# Autodesk Inventor assembly: sip_n_puff_assembly
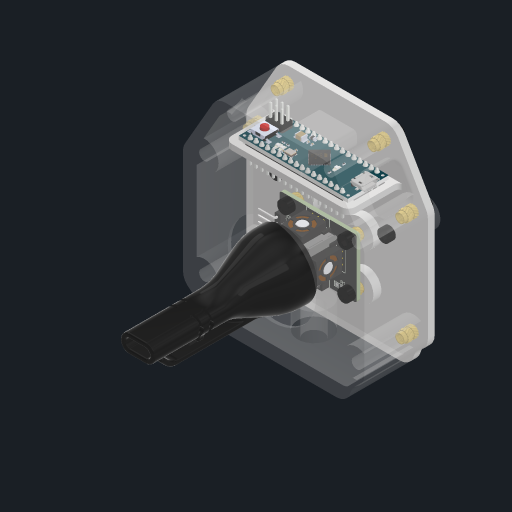
[picture p0: Inventor's stored thumbnail of the model, 512x512]
Saved by Autodesk Inventor 2024 (Build 280153000, 153)
## iProperties
Created: 2025-03-05
Part Number: sip_n_puff_assembly
Document SubType Name: Assembly
Designer: colel
Author: colel
## Documents named in this file (10)
- C:\Users\colel\OneDrive\Desktop\Desktop Folders\Dorm Projects\sip_n_puff_project\sip_n_puff_assembly.iam
- C:\Users\colel\OneDrive\Desktop\Desktop Folders\Dorm Projects\sip_n_puff_project\full_joystick.iam
- C:\Users\colel\OneDrive\Desktop\Desktop Folders\Dorm Projects\sip_n_puff_project\3mm x 6mmL screw.ipt
- C:\Users\colel\OneDrive\Desktop\Desktop Folders\Dorm Projects\sip_n_puff_project\Insert M3 D5 L5mm.ipt
- C:\Users\colel\OneDrive\Desktop\Desktop Folders\Dorm Projects\sip_n_puff_project\mouthpiece.ipt
- C:\Users\colel\OneDrive\Desktop\Desktop Folders\Dorm Projects\sip_n_puff_project\6X6X4.3_BUTTON.ipt
- C:\Users\colel\OneDrive\Desktop\Desktop Folders\Dorm Projects\sip_n_puff_project\Sip_n_box.ipt
- C:\Users\colel\OneDrive\Desktop\Desktop Folders\Dorm Projects\sip_n_puff_project\sip_n_cap.ipt
- C:\Users\colel\OneDrive\Desktop\Desktop Folders\Dorm Projects\sip_n_puff_project\pressure_housing.ipt
- C:\Users\colel\OneDrive\Desktop\Desktop Folders\Dorm Projects\Arduino Stuff\ARDUINO MICRO.iam
## Components (31 placed, 9 different names)
1. full_joystick:1 [sub-assembly] — Mate:1, Mate:2, Mate:3, Mate:4, Mate:5, Mate:6, Mate:7, Mate:8, Mate:10, Mate:14, Mate:15, Mate:16, Mate:21, Mate:22, Tangent:1
2. 3mm x 6mmL screw:1 — Mate:1, Mate:2, Mate:12
3. 3mm x 6mmL screw:2 — Mate:7, Mate:8, Mate:9
4. 3mm x 6mmL screw:3 — Mate:5, Mate:6, Mate:13
5. 3mm x 6mmL screw:4 — Mate:3, Mate:4, Mate:11
6. Insert M3 D5 L5mm:1 — Mate:9, Mate:10
7. Insert M3 D5 L5mm:2 — Mate:12, Mate:16, Mate:25
8. Insert M3 D5 L5mm:3 — Mate:13, Mate:15, Mate:24, Mate:26
9. Insert M3 D5 L5mm:4 — Mate:11, Mate:14
10. mouthpiece:1 — Mate:19, Mate:20, Mate:21, Mate:22, Tangent:1, Mate:23
11. 6X6X4.3_BUTTON:1 — Mate:19, Mate:20, Mate:23
12. Sip_n_box:1 — Mate:24, Mate:25, Mate:26, Mate:36, Mate:37, Mate:44, Mate:45, Mate:46, Mate:47, Mate:49, Mate:50, Mate:51, Mate:52, Mate:53, Mate:54, Mate:55, Mate:56, Mate:57, Mate:58, Mate:59, Mate:60, Mate:65, Mate:66, Mate:67, Mate:68, Mate:69
13. sip_n_cap:1 — Mate:30, Flush:1, Mate:31, Flush:2, Mate:32, Flush:3, Mate:33, Flush:4, Mate:34, Flush:5, Mate:35, Flush:6, Mate:69
14. Insert M3 D5 L5mm:7 — Mate:33, Flush:4, Mate:36
15. Insert M3 D5 L5mm:8 — Mate:34, Flush:5
16. Insert M3 D5 L5mm:9 — Mate:35, Flush:6
17. Insert M3 D5 L5mm:10 — Mate:32, Flush:3
18. Insert M3 D5 L5mm:11 — Mate:31, Flush:2
19. Insert M3 D5 L5mm:12 — Mate:30, Flush:1, Mate:37
20. Insert M3 D5 L5mm:13 — Mate:62, Flush:8
21. Insert M3 D5 L5mm:16 — Mate:61, Flush:7
22. 3mm x 6mmL screw:5 — Mate:46, Mate:47, Mate:63
23. 3mm x 6mmL screw:6 — Mate:44, Mate:45, Mate:64
24. 3mm x 6mmL screw:7 — Mate:49, Mate:50
25. 3mm x 6mmL screw:8 — Mate:55, Mate:56
26. 3mm x 6mmL screw:9 — Mate:57, Mate:58
27. 3mm x 6mmL screw:10 — Mate:59, Mate:60
28. 3mm x 6mmL screw:11 — Mate:53, Mate:54
29. 3mm x 6mmL screw:12 — Mate:51, Mate:52
30. pressure_housing:1 — Mate:61, Flush:7, Mate:62, Flush:8, Mate:63, Mate:64, Mate:65
31. ARDUINO MICRO:1 [sub-assembly] — Mate:66, Mate:67, Mate:68
## Relationships (66: Mate 57, Flush 8, Tangent 1)
- Mate:1: full_joystick:1 ↔ 3mm x 6mmL screw:1
- Mate:2: full_joystick:1 ↔ 3mm x 6mmL screw:1
- Mate:3: full_joystick:1 ↔ 3mm x 6mmL screw:4
- Mate:4: full_joystick:1 ↔ 3mm x 6mmL screw:4
- Mate:5: full_joystick:1 ↔ 3mm x 6mmL screw:3
- Mate:6: full_joystick:1 ↔ 3mm x 6mmL screw:3
- Mate:7: full_joystick:1 ↔ 3mm x 6mmL screw:2
- Mate:8: full_joystick:1 ↔ 3mm x 6mmL screw:2
- Mate:9: 3mm x 6mmL screw:2 ↔ Insert M3 D5 L5mm:1
- Mate:10: full_joystick:1 ↔ Insert M3 D5 L5mm:1
- Mate:11: 3mm x 6mmL screw:4 ↔ Insert M3 D5 L5mm:4
- Mate:12: 3mm x 6mmL screw:1 ↔ Insert M3 D5 L5mm:2
- Mate:13: 3mm x 6mmL screw:3 ↔ Insert M3 D5 L5mm:3
- Mate:14: full_joystick:1 ↔ Insert M3 D5 L5mm:4
- Mate:15: full_joystick:1 ↔ Insert M3 D5 L5mm:3
- Mate:16: full_joystick:1 ↔ Insert M3 D5 L5mm:2
- Mate:19 (0.25 mm): mouthpiece:1 ↔ 6X6X4.3_BUTTON:1
- Mate:20 (0.25 mm): mouthpiece:1 ↔ 6X6X4.3_BUTTON:1
- Mate:21 (0.25 mm): full_joystick:1 ↔ mouthpiece:1
- Mate:22 (0.25 mm): full_joystick:1 ↔ mouthpiece:1
- Tangent:1: full_joystick:1 ↔ mouthpiece:1
- Mate:23: mouthpiece:1 ↔ 6X6X4.3_BUTTON:1
- Mate:24: Insert M3 D5 L5mm:3 ↔ Sip_n_box:1
- Mate:25: Insert M3 D5 L5mm:2 ↔ Sip_n_box:1
- Mate:26: Insert M3 D5 L5mm:3 ↔ Sip_n_box:1
- Mate:30: sip_n_cap:1 ↔ Insert M3 D5 L5mm:12
- Flush:1: sip_n_cap:1 ↔ Insert M3 D5 L5mm:12
- Mate:31: sip_n_cap:1 ↔ Insert M3 D5 L5mm:11
- Flush:2: sip_n_cap:1 ↔ Insert M3 D5 L5mm:11
- Mate:32: sip_n_cap:1 ↔ Insert M3 D5 L5mm:10
- Flush:3: sip_n_cap:1 ↔ Insert M3 D5 L5mm:10
- Mate:33: sip_n_cap:1 ↔ Insert M3 D5 L5mm:7
- Flush:4: sip_n_cap:1 ↔ Insert M3 D5 L5mm:7
- Mate:34: sip_n_cap:1 ↔ Insert M3 D5 L5mm:8
- Flush:5: sip_n_cap:1 ↔ Insert M3 D5 L5mm:8
- Mate:35: sip_n_cap:1 ↔ Insert M3 D5 L5mm:9
- Flush:6: sip_n_cap:1 ↔ Insert M3 D5 L5mm:9
- Mate:36: Sip_n_box:1 ↔ Insert M3 D5 L5mm:7
- Mate:37: Sip_n_box:1 ↔ Insert M3 D5 L5mm:12
- Mate:44: Sip_n_box:1 ↔ 3mm x 6mmL screw:6
- Mate:45: Sip_n_box:1 ↔ 3mm x 6mmL screw:6
- Mate:46: Sip_n_box:1 ↔ 3mm x 6mmL screw:5
- Mate:47: Sip_n_box:1 ↔ 3mm x 6mmL screw:5
- Mate:49: Sip_n_box:1 ↔ 3mm x 6mmL screw:7
- Mate:50: Sip_n_box:1 ↔ 3mm x 6mmL screw:7
- Mate:51: Sip_n_box:1 ↔ 3mm x 6mmL screw:12
- Mate:52: Sip_n_box:1 ↔ 3mm x 6mmL screw:12
- Mate:53: Sip_n_box:1 ↔ 3mm x 6mmL screw:11
- Mate:54: Sip_n_box:1 ↔ 3mm x 6mmL screw:11
- Mate:55: Sip_n_box:1 ↔ 3mm x 6mmL screw:8
- Mate:56: Sip_n_box:1 ↔ 3mm x 6mmL screw:8
- Mate:57: Sip_n_box:1 ↔ 3mm x 6mmL screw:9
- Mate:58: Sip_n_box:1 ↔ 3mm x 6mmL screw:9
- Mate:59: Sip_n_box:1 ↔ 3mm x 6mmL screw:10
- Mate:60: Sip_n_box:1 ↔ 3mm x 6mmL screw:10
- Mate:61: Insert M3 D5 L5mm:16 ↔ pressure_housing:1
- Flush:7: Insert M3 D5 L5mm:16 ↔ pressure_housing:1
- Mate:62: Insert M3 D5 L5mm:13 ↔ pressure_housing:1
- Flush:8: Insert M3 D5 L5mm:13 ↔ pressure_housing:1
- Mate:63: 3mm x 6mmL screw:5 ↔ pressure_housing:1
- Mate:64: 3mm x 6mmL screw:6 ↔ pressure_housing:1
- Mate:65: Sip_n_box:1 ↔ pressure_housing:1
- Mate:66 (0.5 mm): Sip_n_box:1 ↔ ARDUINO MICRO:1
- Mate:67 (0.5 mm): Sip_n_box:1 ↔ ARDUINO MICRO:1
- Mate:68: Sip_n_box:1 ↔ ARDUINO MICRO:1
- Mate:69: Sip_n_box:1 ↔ sip_n_cap:1
